# Autodesk Inventor assembly: Skrzydło
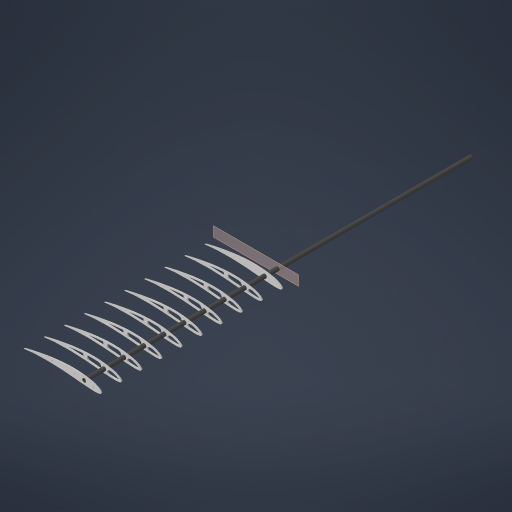
[picture p0: Inventor's stored thumbnail of the model, 512x512]
Saved by Autodesk Inventor 2023 (Build 270158000, 158)
## iProperties
Created: 2022-11-20
Part Number: Skrzydło
Document SubType Name: Assembly
Designer: szykr
Author: szykr
## Documents named in this file (5)
- D:\Folder Instalacyjny\GitHub Pliki\Solaris\model\Skrzydło.iam
- D:\Folder Instalacyjny\GitHub Pliki\Solaris\model\Żebro Montaż.ipt
- D:\Folder Instalacyjny\GitHub Pliki\Solaris\model\Wingspar metrowy.ipt
- D:\Folder Instalacyjny\GitHub Pliki\Solaris\model\Żebro Default.ipt
- D:\Folder Instalacyjny\GitHub Pliki\Solaris\model\Żebro_Kadłub.ipt
## Components (11 placed, 4 different names)
1. Żebro Montaż:1 — Mate:1, Symmetry:1, Insert:3
2. Wingspar metrowy:1 — Mate:1, Symmetry:1, Insert:2
3. Żebro_Kadłub:1 — Insert:2
4. Żebro Default:1 — Insert:3
5. Żebro Default:2
6. Żebro Default:3
7. Żebro Default:4
8. Żebro Default:5
9. Żebro Default:6
10. Żebro Default:7
11. Żebro Default:8
## Component patterns: (8 elements, first: Żebro Default:1)
## Relationships (4: Insert 2, Mate 1, Symmetry 1)
- Mate:1: Żebro Montaż:1 ↔ Wingspar metrowy:1
- Symmetry:1: Żebro Montaż:1 ↔ Wingspar metrowy:1
- Insert:2 (467 mm): Wingspar metrowy:1 ↔ Żebro_Kadłub:1
- Insert:3 (51.8889 mm): Żebro Montaż:1 ↔ Żebro Default:1
## Named parameters: rozstaw_zeber = 51.88889 mm, ilosc_zeber_h = 10, ilosc_zeber = 8, szerokosc_kadluba = 60 mm
